# Autodesk Inventor assembly: 42146-33
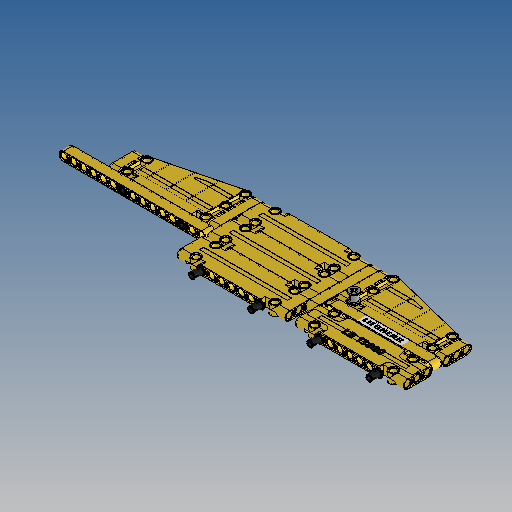
[picture p0: Inventor's stored thumbnail of the model, 512x512]
Saved by Autodesk Inventor 2025 (Build 290162010, 162A)
## iProperties
Created: 2024-12-06
Part Number: 42146-33
Material: Generisch
Document SubType Name: Assembly
Designer: hp.muther
Author: hp.muther
## Documents named in this file (10)
- D:\Inventor\Projekte\Muther\LEGO Technic\LEGO Technik - Raupenkran LR 13000 (42146)\42146-33.iam
- D:\Inventor\Projekte\Muther\LEGO Technic\LEGO Pieces\Paneelen\15458-Yellow.ipt
- D:\Inventor\Projekte\Muther\LEGO Technic\LEGO Pieces\Pin's\2780-Black.ipt
- D:\Inventor\Projekte\Muther\LEGO Technic\LEGO Technik - Raupenkran LR 13000 (42146)\42146_15458_2.ipt
- D:\Inventor\Projekte\Muther\LEGO Technic\LEGO Technik - Raupenkran LR 13000 (42146)\42146_32525_1.ipt
- D:\Inventor\Projekte\Muther\LEGO Technic\LEGO Pieces\Lochbalken\32524-Yellow.ipt
- D:\Inventor\Projekte\Muther\LEGO Technic\LEGO Pieces\Pin's\6558-Blue.ipt
- D:\Inventor\Projekte\Muther\LEGO Technic\LEGO Pieces\Paneelen\18945-Yellow.ipt
- D:\Inventor\Projekte\Muther\LEGO Technic\LEGO Pieces\Pin's\32054-LtBluishGray.ipt
- D:\Inventor\Projekte\Muther\LEGO Technic\LEGO Pieces\Lochbalken\32278-Yellow.ipt
## Components (26 placed, 9 different names)
1. 15458-Yellow:1 — Einfügen:3, Einfügen:4, Einfügen:14, Passend:4
2. 2780-Black:1 — Einfügen:3
3. 2780-Black:2 — Einfügen:4
4. 42146_15458_2:1 — Einfügen:8, Passend:2, Einfügen:22, Einfügen:23
5. 42146_32525_1:1 — Einfügen:1, Einfügen:2, Einfügen:6, Einfügen:8
6. 32524-Yellow:1 — Einfügen:9, Passend:3, Einfügen:16
7. 6558-Blue:1 — Einfügen:1, Passend:2
8. 6558-Blue:2 — Einfügen:2, Passend:1
9. 6558-Blue:3 — Einfügen:7, Passend:3, Passend:6
10. 6558-Blue:4 — Einfügen:5
11. 18945-Yellow:1 — Einfügen:5, Einfügen:6, Einfügen:7, Passend:1, Einfügen:9, Einfügen:24
12. 15458-Yellow:2 — Einfügen:14, Einfügen:15, Passend:5, Passend:6, Passend:7
13. 2780-Black:3 — Passend:4
14. 2780-Black:4
15. 15458-Yellow:3 — Einfügen:15, Einfügen:16, Einfügen:21
16. 2780-Black:5 — Passend:5
17. 2780-Black:6
18. 18945-Yellow:2 — Einfügen:17, Einfügen:18, Einfügen:19, Einfügen:20, Einfügen:21, Einfügen:25
19. 2780-Black:7 — Einfügen:19
20. 2780-Black:8 — Einfügen:20, Passend:8
21. 2780-Black:9 — Einfügen:17
22. 2780-Black:10 — Einfügen:18, Passend:7
23. 2780-Black:11 — Einfügen:22
24. 2780-Black:12 — Einfügen:23
25. 32054-LtBluishGray:1 — Einfügen:24
26. 32278-Yellow:1 — Einfügen:25, Passend:8
## Relationships (33: Insert 25, Mate 8)
- Einfügen:1 [Insert]: 42146_32525_1:1 ↔ 6558-Blue:1
- Einfügen:2 [Insert]: 42146_32525_1:1 ↔ 6558-Blue:2
- Einfügen:3 [Insert]: 15458-Yellow:1 ↔ 2780-Black:1
- Einfügen:4 [Insert]: 15458-Yellow:1 ↔ 2780-Black:2
- Einfügen:5 [Insert]: 6558-Blue:4 ↔ 18945-Yellow:1
- Einfügen:6 [Insert]: 42146_32525_1:1 ↔ 18945-Yellow:1
- Einfügen:7 [Insert]: 6558-Blue:3 ↔ 18945-Yellow:1
- Passend:1 [Mate]: 6558-Blue:2 ↔ 18945-Yellow:1
- Einfügen:8 [Insert]: 42146_15458_2:1 ↔ 42146_32525_1:1
- Passend:2 [Mate]: 42146_15458_2:1 ↔ 6558-Blue:1
- Einfügen:9 [Insert]: 32524-Yellow:1 ↔ 18945-Yellow:1
- Passend:3 [Mate]: 32524-Yellow:1 ↔ 6558-Blue:3
- [Insert]: 15458-Yellow:2 ↔ 2780-Black:3
- [Insert]: 15458-Yellow:2 ↔ 2780-Black:4
- [Insert]: 15458-Yellow:3 ↔ 2780-Black:5
- [Insert]: 15458-Yellow:3 ↔ 2780-Black:6
- Einfügen:14 [Insert]: 15458-Yellow:1 ↔ 15458-Yellow:2
- Einfügen:15 [Insert]: 15458-Yellow:2 ↔ 15458-Yellow:3
- Passend:4 [Mate]: 15458-Yellow:1 ↔ 2780-Black:3
- Passend:5 [Mate]: 15458-Yellow:2 ↔ 2780-Black:5
- Einfügen:16 [Insert]: 32524-Yellow:1 ↔ 15458-Yellow:3
- Passend:6 [Mate]: 6558-Blue:3 ↔ 15458-Yellow:2
- Einfügen:17 [Insert]: 18945-Yellow:2 ↔ 2780-Black:9
- Einfügen:18 [Insert]: 18945-Yellow:2 ↔ 2780-Black:10
- Einfügen:19 [Insert]: 18945-Yellow:2 ↔ 2780-Black:7
- Einfügen:20 [Insert]: 18945-Yellow:2 ↔ 2780-Black:8
- Einfügen:21 [Insert]: 15458-Yellow:3 ↔ 18945-Yellow:2
- Passend:7 [Mate]: 15458-Yellow:2 ↔ 2780-Black:10
- Einfügen:22 [Insert]: 42146_15458_2:1 ↔ 2780-Black:11
- Einfügen:23 [Insert]: 42146_15458_2:1 ↔ 2780-Black:12
- Einfügen:24 [Insert]: 18945-Yellow:1 ↔ 32054-LtBluishGray:1
- Einfügen:25 [Insert]: 18945-Yellow:2 ↔ 32278-Yellow:1
- Passend:8 [Mate]: 2780-Black:8 ↔ 32278-Yellow:1
## Named parameters: d12_d2 = 0 mm, d13_d3 = 0 mm, d14_d2 = 0 mm, d15_d3 = 0 mm
